# Autodesk Inventor assembly: trucks
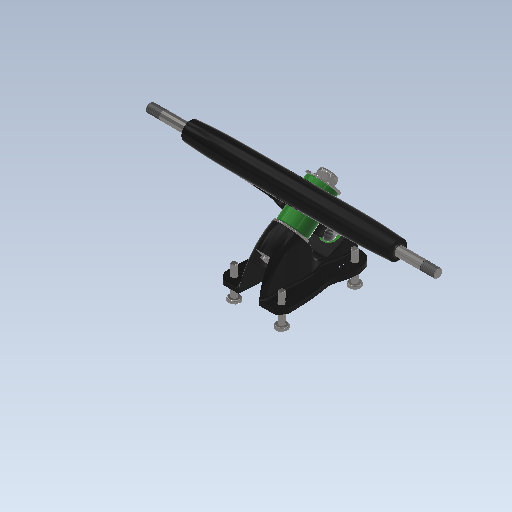
[picture p0: Inventor's stored thumbnail of the model, 512x512]
Saved by Autodesk Inventor 2020.1 (Build 241239000, 239)
## iProperties
Created: 2018-11-22
Part Number: trucks
Document SubType Name: Assembly
Designer: Petar
Mass: 345.903 g
Surface Area: 498.588 cm^2
Volume: 134.836 cm^3
Density: 2.56536 g/cm^3
Author: Petar
## Documents named in this file (10)
- D:\OMG\E-Board\CAD\Inventor\trucks.iam
- D:\OMG\E-Board\CAD\Inventor\Trucks\trucks_base.ipt
- D:\OMG\E-Board\CAD\Inventor\Trucks\trucks_bushing.ipt
- D:\OMG\E-Board\CAD\Inventor\Trucks\trucks_kingpin_nut.ipt
- D:\OMG\E-Board\CAD\Inventor\Trucks\trucks_washer.ipt
- D:\OMG\E-Board\CAD\Inventor\Trucks\trucks_pivot_cup.ipt
- D:\OMG\E-Board\CAD\Inventor\Trucks\trucks_kingpin.ipt
- D:\OMG\E-Board\CAD\Inventor\Trucks\trucks_hanger.ipt
- D:\OMG\E-Board\CAD\Inventor\Trucks\pan_head_screw.ipt
- D:\OMG\E-Board\CAD\Inventor\Trucks\speed_washer.ipt
## Components (15 placed, 9 different names)
1. trucks_bushing:2 — Insert:5, Insert:14
2. trucks_kingpin_nut:1 — Insert:8
3. trucks_washer:1 — Insert:5, Insert:8
4. trucks_base:1 — Insert:9, Insert:10, Insert:16, Insert:17, Insert:18, Insert:19, Insert:20
5. trucks_pivot_cup:1 — Insert:9, Insert:12
6. trucks_kingpin:1 — Insert:10
7. trucks_hanger:1 — Insert:12, Insert:14, Insert:21, Insert:22
8. trucks_washer:2 — Insert:15, Insert:16
9. trucks_bushing:3 — Insert:15
10. pan_head_screw:1 — Insert:17
11. pan_head_screw:2 — Insert:20
12. pan_head_screw:3 — Insert:19
13. pan_head_screw:4 — Insert:18
14. speed_washer:1 — Insert:22
15. speed_washer:2 — Insert:21
## Relationships (14: Insert 14)
- Insert:5: trucks_bushing:2 ↔ trucks_washer:1
- Insert:8: trucks_kingpin_nut:1 ↔ trucks_washer:1
- Insert:9: trucks_base:1 ↔ trucks_pivot_cup:1
- Insert:10: trucks_base:1 ↔ trucks_kingpin:1
- Insert:12: trucks_pivot_cup:1 ↔ trucks_hanger:1
- Insert:14: trucks_bushing:2 ↔ trucks_hanger:1
- Insert:15: trucks_washer:2 ↔ trucks_bushing:3
- Insert:16: trucks_base:1 ↔ trucks_washer:2
- Insert:17 (11.855 mm): trucks_base:1 ↔ pan_head_screw:1
- Insert:18 (11.855 mm): trucks_base:1 ↔ pan_head_screw:4
- Insert:19 (11.855 mm): trucks_base:1 ↔ pan_head_screw:3
- Insert:20 (11.855 mm): trucks_base:1 ↔ pan_head_screw:2
- Insert:21: trucks_hanger:1 ↔ speed_washer:2
- Insert:22: trucks_hanger:1 ↔ speed_washer:1
